# Autodesk Inventor assembly: antenna_unit
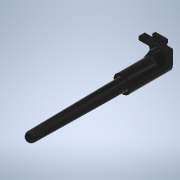
[picture p0: Inventor's stored thumbnail of the model, 180x180]
Saved by Autodesk Inventor 2020 (Build 240168000, 168)
## iProperties
Created: 2021-06-17
Part Number: antenna_unit
Document SubType Name: Assembly
Designer: masato
Mass: 11.8411 g
Surface Area: 44.2768 cm^2
Volume: 8.30955 cm^3
Density: 1.425 g/cm^3
Author: masato
## Documents named in this file (4)
- C:\Users\Masato\Documents\Inventor\CIT Brains_Inventor\コックピット\OpenPlatform_ver3_0\上半身\コックピット\Antenna_unit.iam
- C:\Users\Masato\Documents\Inventor\CIT Brains_Inventor\コックピット\OpenPlatform_ver3_0\上半身\コックピット\antenna.ipt
- C:\Users\Masato\Documents\Inventor\CIT Brains_Inventor\コックピット\OpenPlatform_ver3_0\上半身\コックピット\Antenna_frame_01.ipt
- C:\Users\Masato\Documents\Inventor\CIT Brains_Inventor\コックピット\OpenPlatform_ver3_0\上半身\コックピット\Antenna_cover_01.ipt
## Components (3 placed, 3 different names)
1. Antenna_frame_01:1 — 挿入:1, 挿入:2, 挿入:3
2. Antenna:1 — 挿入:1
3. Antenna_cover_01:1 — 挿入:2, 挿入:3
## Relationships (3: Insert 3)
- 挿入:1 [Insert]: Antenna_frame_01:1 ↔ Antenna:1
- 挿入:2 [Insert]: Antenna_frame_01:1 ↔ Antenna_cover_01:1
- 挿入:3 [Insert]: Antenna_frame_01:1 ↔ Antenna_cover_01:1
